# Autodesk Inventor assembly: gas
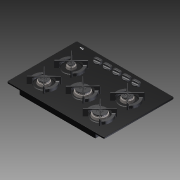
[picture p0: Inventor's stored thumbnail of the model, 180x180]
Saved by Autodesk Inventor 2015 (Build 190159000, 159)
## iProperties
Created: 2015-10-18
Part Number: gas
Document SubType Name: Assembly
Designer: omae
Author: omae
## Documents named in this file (2)
- C:\Users\omae\Desktop\研究室\論文・資料\ROS\kitchen\stl\gas.iam
- C:\Users\omae\Desktop\研究室\論文・資料\ROS\kitchen\tool\konro.iam
## Components (1 placed, 1 different names)
1. konro:1 [sub-assembly] — フラッシュ:1, フラッシュ:2, フラッシュ:3
## Relationships (3: Flush 3)
- フラッシュ:1 [Flush]: konro:1
- フラッシュ:2 [Flush]: konro:1
- フラッシュ:3 [Flush]: konro:1
